# Autodesk Inventor assembly: Assembly2
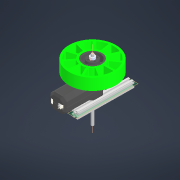
[picture p0: Inventor's stored thumbnail of the model, 180x180]
Saved by Autodesk Inventor 2022 (Build 260153000, 153)
## iProperties
Created: 2021-10-09
Part Number: Assembly2
Document SubType Name: Assembly
Designer: zehrab
Author: zehrab
## Documents named in this file (12)
- C:\Users\zehrab\Documents\GitHub\ComputerAidedDesign\2021-22\FTC\#13822 Robovikes\Duck Carousel\Assembly2.iam
- C:\Users\zehrab\Documents\GitHub\ComputerAidedDesign\2021-22\FTC\#13822 Robovikes\Duck Carousel\Carousel Base.ipt
- C:\Users\zehrab\Documents\GitHub\ComputerAidedDesign\2021-22\FTC\#13822 Robovikes\Duck Carousel\Carousel.ipt
- C:\Users\zehrab\Documents\GitHub\ComputerAidedDesign\2021-22\FTC\#13822 Robovikes\Duck Carousel\am-4510 Rubber Duck.ipt
- C:\Users\zehrab\Documents\GitHub\ComputerAidedDesign\2021-22\FTC\#13822 Robovikes\Duck Carousel\REV-41-1349.ipt
- C:\Users\zehrab\Documents\GitHub\ComputerAidedDesign\2021-22\FTC\#13822 Robovikes\Duck Carousel\am-4538 4IN 5mm Hex Compliant Wheel.ipt
- C:\Users\zehrab\Documents\GitHub\ComputerAidedDesign\2021-22\FTC\#13822 Robovikes\Duck Carousel\Slim Shaft Collar - 10 Pack.ipt
- C:\Users\zehrab\Documents\GitHub\ComputerAidedDesign\2021-22\FTC\#13822 Robovikes\Duck Carousel\3mm Spacer - 16 Pack.ipt
- C:\Users\zehrab\Documents\GitHub\ComputerAidedDesign\2021-22\FTC\#13822 Robovikes\Duck Carousel\REV-41-1300.ipt
- C:\Users\zehrab\Documents\GitHub\ComputerAidedDesign\2021-22\FTC\#13822 Robovikes\Duck Carousel\REV-41-1433.ipt
- C:\Users\zehrab\Documents\GitHub\ComputerAidedDesign\2021-22\FTC\#13822 Robovikes\Duck Carousel\15mm Extrusion - 120mm - 90° Ends - 2 Pack.ipt
- C:\Users\zehrab\Documents\GitHub\ComputerAidedDesign\2021-22\FTC\#13822 Robovikes\Duck Carousel\M3 x 8mm Hex Cap Screws - 100 Pack.ipt
## Components (17 placed, 11 different names)
1. Carousel Base:1 — Mate:1, Flush:1
2. Carousel:1 — Mate:1, Flush:1, Mate:2, Tangent:1, Angle:7
3. am-4510 Rubber Duck:1 — Mate:2
4. REV-41-1349:1 — Mate:10, Mate:11, Mate:12, Mate:13, Mate:14, Mate:17, Mate:19
5. am-4538 4IN 5mm Hex Compliant Wheel:1 — Mate:12, Tangent:1, Angle:7, Mate:15, Mate:16
6. Slim Shaft Collar - 10 Pack:1 — Mate:10, Angle:6, Mate:15
7. Slim Shaft Collar - 10 Pack:2 — Mate:11, Angle:6
8. 3mm Spacer - 16 Pack:1 — Mate:13, Mate:14, Mate:16, Mate:18
9. REV-41-1300:1 — Mate:17, Mate:18, Mate:20, Angle:8, Mate:22, Mate:24, Mate:25, Mate:26, Mate:27
10. REV-41-1433:1 — Mate:19, Mate:20, Angle:8, Mate:21, Mate:23, Mate:31, Mate:33
11. 15mm Extrusion - 120mm - 90° Ends - 2 Pack:1 — Mate:21, Mate:22, Flush:5, Symmetry:1, Mate:28, Mate:29
12. M3 x 8mm Hex Cap Screws - 100 Pack:1 — Flush:2, Mate:23, Mate:24
13. M3 x 8mm Hex Cap Screws - 100 Pack:2 — Flush:2, Flush:3, Mate:25
14. M3 x 8mm Hex Cap Screws - 100 Pack:3 — Flush:3, Flush:4, Mate:26
15. M3 x 8mm Hex Cap Screws - 100 Pack:4 — Flush:4, Mate:27
16. M3 x 8mm Hex Cap Screws - 100 Pack:5 — Mate:28, Mate:32, Mate:33
17. M3 x 8mm Hex Cap Screws - 100 Pack:6 — Mate:29, Mate:30, Mate:31
## Relationships (36: Mate 26, Flush 5, Angle 3, Tangent 1, Symmetry 1)
- Mate:1: Carousel Base:1 ↔ Carousel:1
- Flush:1: Carousel Base:1 ↔ Carousel:1
- Mate:2: Carousel:1 ↔ am-4510 Rubber Duck:1
- Mate:10: REV-41-1349:1 ↔ Slim Shaft Collar - 10 Pack:1
- Mate:11: REV-41-1349:1 ↔ Slim Shaft Collar - 10 Pack:2
- Angle:6 (0 deg): Slim Shaft Collar - 10 Pack:1 ↔ Slim Shaft Collar - 10 Pack:2
- Mate:12: REV-41-1349:1 ↔ am-4538 4IN 5mm Hex Compliant Wheel:1
- Tangent:1: Carousel:1 ↔ am-4538 4IN 5mm Hex Compliant Wheel:1
- Angle:7 (0 deg): Carousel:1 ↔ am-4538 4IN 5mm Hex Compliant Wheel:1
- Mate:13: REV-41-1349:1 ↔ 3mm Spacer - 16 Pack:1
- Mate:14: REV-41-1349:1 ↔ 3mm Spacer - 16 Pack:1
- Mate:15: am-4538 4IN 5mm Hex Compliant Wheel:1 ↔ Slim Shaft Collar - 10 Pack:1
- Mate:16: am-4538 4IN 5mm Hex Compliant Wheel:1 ↔ 3mm Spacer - 16 Pack:1
- Mate:17: REV-41-1349:1 ↔ REV-41-1300:1
- Mate:18: 3mm Spacer - 16 Pack:1 ↔ REV-41-1300:1
- Mate:19: REV-41-1349:1 ↔ REV-41-1433:1
- Mate:20: REV-41-1300:1 ↔ REV-41-1433:1
- Angle:8 (180 deg): REV-41-1300:1 ↔ REV-41-1433:1
- Mate:21: REV-41-1433:1 ↔ 15mm Extrusion - 120mm - 90° Ends - 2 Pack:1
- Mate:22: REV-41-1300:1 ↔ 15mm Extrusion - 120mm - 90° Ends - 2 Pack:1
- Flush:2: M3 x 8mm Hex Cap Screws - 100 Pack:1 ↔ M3 x 8mm Hex Cap Screws - 100 Pack:2
- Flush:3: M3 x 8mm Hex Cap Screws - 100 Pack:2 ↔ M3 x 8mm Hex Cap Screws - 100 Pack:3
- Flush:4: M3 x 8mm Hex Cap Screws - 100 Pack:3 ↔ M3 x 8mm Hex Cap Screws - 100 Pack:4
- Mate:23: REV-41-1433:1 ↔ M3 x 8mm Hex Cap Screws - 100 Pack:1
- Mate:24: REV-41-1300:1 ↔ M3 x 8mm Hex Cap Screws - 100 Pack:1
- Mate:25: REV-41-1300:1 ↔ M3 x 8mm Hex Cap Screws - 100 Pack:2
- Mate:26: REV-41-1300:1 ↔ M3 x 8mm Hex Cap Screws - 100 Pack:3
- Mate:27: REV-41-1300:1 ↔ M3 x 8mm Hex Cap Screws - 100 Pack:4
- Flush:5: 15mm Extrusion - 120mm - 90° Ends - 2 Pack:1
- Symmetry:1: 15mm Extrusion - 120mm - 90° Ends - 2 Pack:1
- Mate:28: 15mm Extrusion - 120mm - 90° Ends - 2 Pack:1 ↔ M3 x 8mm Hex Cap Screws - 100 Pack:5
- Mate:29: 15mm Extrusion - 120mm - 90° Ends - 2 Pack:1 ↔ M3 x 8mm Hex Cap Screws - 100 Pack:6
- Mate:30: M3 x 8mm Hex Cap Screws - 100 Pack:6
- Mate:31: REV-41-1433:1 ↔ M3 x 8mm Hex Cap Screws - 100 Pack:6
- Mate:32: M3 x 8mm Hex Cap Screws - 100 Pack:5
- Mate:33: REV-41-1433:1 ↔ M3 x 8mm Hex Cap Screws - 100 Pack:5
